# Autodesk Inventor assembly: ensambleSoporteMarcador
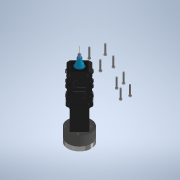
[picture p0: Inventor's stored thumbnail of the model, 180x180]
Saved by Autodesk Inventor 2021.5 (Build 255421000, 421)
## iProperties
Created: 2024-11-20
Part Number: ensambleSoporteMarcador
Document SubType Name: Assembly
Designer: Joho_
Mass: 142.225 g
Surface Area: 565.356 cm^2
Volume: 144.665 cm^3
Density: 0.983135 g/cm^3
Author: Joho_
## Documents named in this file (6)
- C:\Users\Joho_\Desktop\semestreN\robotica\laboratorios\lab01\CADs\ensambleSoporteMarcador.iam
- C:\Users\Joho_\Desktop\semestreN\robotica\laboratorios\lab01\CADs\flancheDeMontaje.ipt
- C:\Users\Joho_\Desktop\semestreN\robotica\laboratorios\lab01\CADs\baseSoporte.ipt
- C:\Users\Joho_\Desktop\semestreN\robotica\laboratorios\lab01\CADs\acople.ipt
- C:\Users\Joho_\Desktop\semestreN\robotica\laboratorios\lab01\CADs\marcador.ipt
- C:\Users\Joho_\Desktop\semestreN\robotica\laboratorios\lab01\CADs\tonrilloM3x20mm.ipt
## Components (13 placed, 5 different names)
1. flancheDeMontaje:1 — Nivelación:1, Nivelación:2, Nivelación:3, Coincidencia:1, Coincidencia:2, Coincidencia:3
2. baseSoporte:1 — Coincidencia:1, Coincidencia:2, Coincidencia:3, Coincidencia:4, Coincidencia:5, Coincidencia:6, Coincidencia:10
3. acople:1 — Coincidencia:4, Coincidencia:5, Coincidencia:6, Coincidencia:7, Coincidencia:8, Nivelación:4, Coincidencia:9, Nivelación:5
4. acople:2 — Coincidencia:9, Coincidencia:10, Nivelación:5
5. marcador:1 — Coincidencia:7, Coincidencia:8, Nivelación:4
6. tonrilloM3x20mm:1
7. tonrilloM3x20mm:2
8. tonrilloM3x20mm:3
9. tonrilloM3x20mm:4
10. tonrilloM3x20mm:5
11. tonrilloM3x20mm:6
12. tonrilloM3x20mm:7
13. tonrilloM3x20mm:8
## Relationships (15: Mate 10, Flush 5)
- Nivelación:1 [Flush]: flancheDeMontaje:1
- Nivelación:2 [Flush]: flancheDeMontaje:1
- Nivelación:3 [Flush]: flancheDeMontaje:1
- Coincidencia:1 [Mate]: flancheDeMontaje:1 ↔ baseSoporte:1
- Coincidencia:2 [Mate]: flancheDeMontaje:1 ↔ baseSoporte:1
- Coincidencia:3 [Mate]: flancheDeMontaje:1 ↔ baseSoporte:1
- Coincidencia:4 [Mate]: baseSoporte:1 ↔ acople:1
- Coincidencia:5 [Mate]: baseSoporte:1 ↔ acople:1
- Coincidencia:6 [Mate]: baseSoporte:1 ↔ acople:1
- Coincidencia:7 [Mate]: acople:1 ↔ marcador:1
- Coincidencia:8 [Mate]: acople:1 ↔ marcador:1
- Nivelación:4 [Flush]: acople:1 ↔ marcador:1
- Coincidencia:9 [Mate]: acople:1 ↔ acople:2
- Coincidencia:10 [Mate]: baseSoporte:1 ↔ acople:2
- Nivelación:5 [Flush]: acople:1 ↔ acople:2
